# Autodesk Inventor assembly: Assembly1
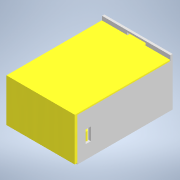
[picture p0: Inventor's stored thumbnail of the model, 180x180]
Saved by Autodesk Inventor 2022.2 (Build 262287000, 287)
## iProperties
Created: 2022-01-19
Part Number: Assembly1
Document SubType Name: Assembly
Designer: samlo
Author: samlo
## Documents named in this file (3)
- D:\Documents\case\bins\Assembly1.iam
- D:\Documents\case\bins\top.ipt
- C:\Users\samlo\OneDrive\Documents\bin v1.ipt
## Components (2 placed, 2 different names)
1. bin v1:1 — Mate:1, Rigid:1
2. top:1 — Mate:1, Rigid:1
## Relationships (2: Mate 1, WeldJoint 1)
- Mate:1: bin v1:1 ↔ top:1
- Rigid:1 [WeldJoint]: bin v1:1 ↔ top:1
